# Autodesk Inventor assembly: 05.01.СБ
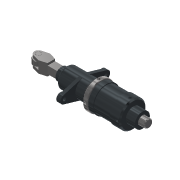
[picture p0: Inventor's stored thumbnail of the model, 180x180]
Saved by Autodesk Inventor 2020 (Build 240168000, 168)
## iProperties
Created: 2018-07-09
Part Number: 05.01.СБ
Material: Типовые
Document SubType Name: Assembly
Designer: MSI-PC
Mass: 2793.56 g
Surface Area: 1144.42 cm^2
Volume: 378.896 cm^3
Density: 7.3729 g/cm^3
Description: Амортизатор
Author: MSI-PC
Title: 05.01.СБ
## Documents named in this file (8)
- C:\Users\Сергей\Desktop\asp\1-Standard Asm\Standard 05.01.СБ.iam
- C:\Users\Сергей\Desktop\Амортизатор_1\05.01.001.ipt
- C:\Users\Сергей\Desktop\Амортизатор_1\05.01.002.ipt
- C:\Users\Сергей\Desktop\Амортизатор_1\05.01.003.ipt
- C:\Users\Сергей\Desktop\Амортизатор_1\05.01.004.ipt
- C:\Users\Сергей\Desktop\Амортизатор_1\05.01.005.ipt
- C:\Users\Сергей\Desktop\Амортизатор_1\05.01.006.ipt
- C:\Users\Сергей\Desktop\Амортизатор_1\05.01.007.ipt
## Components (7 placed, 7 different names)
1. 05.01.001:1 — Совмещение:2, Совмещение:3, Совмещение:4, Совмещение:5, Угол:1
2. 05.01.002:1 — Совмещение:11, Совмещение:12, Совмещение:13, Совмещение:14
3. 05.01.003:1 — Совмещение:6, Совмещение:8, Совмещение:10, Совмещение:11, Совмещение:13
4. 05.01.004:1 — Совмещение:1, Совмещение:2, Заподлицо:1, Совмещение:3
5. 05.01.005:1 — Совмещение:1, Заподлицо:1
6. 05.01.006:1 — Совмещение:9, Совмещение:12, Совмещение:14, Совмещение:15
7. 05.01.007:1 — Совмещение:4, Совмещение:5, Угол:1, Совмещение:6, Совмещение:8, Совмещение:9, Совмещение:10, Совмещение:15
## Relationships (16: Mate 14, Flush 1, Angle 1)
- Совмещение:1 [Mate]: 05.01.004:1 ↔ 05.01.005:1
- Совмещение:2 [Mate]: 05.01.001:1 ↔ 05.01.004:1
- Заподлицо:1 [Flush]: 05.01.004:1 ↔ 05.01.005:1
- Совмещение:3 [Mate]: 05.01.001:1 ↔ 05.01.004:1
- Совмещение:4 [Mate]: 05.01.001:1 ↔ 05.01.007:1
- Совмещение:5 [Mate]: 05.01.001:1 ↔ 05.01.007:1
- Угол:1 [Angle] (0 deg): 05.01.001:1 ↔ 05.01.007:1
- Совмещение:6 [Mate]: 05.01.003:1 ↔ 05.01.007:1
- Совмещение:8 [Mate]: 05.01.003:1 ↔ 05.01.007:1
- Совмещение:9 [Mate]: 05.01.006:1 ↔ 05.01.007:1
- Совмещение:10 [Mate]: 05.01.003:1 ↔ 05.01.007:1
- Совмещение:11 [Mate]: 05.01.002:1 ↔ 05.01.003:1
- Совмещение:12 [Mate]: 05.01.002:1 ↔ 05.01.006:1
- Совмещение:13 [Mate]: 05.01.002:1 ↔ 05.01.003:1
- Совмещение:14 [Mate]: 05.01.002:1 ↔ 05.01.006:1
- Совмещение:15 [Mate] (135 mm): 05.01.006:1 ↔ 05.01.007:1
